# Autodesk Inventor assembly: questionblock
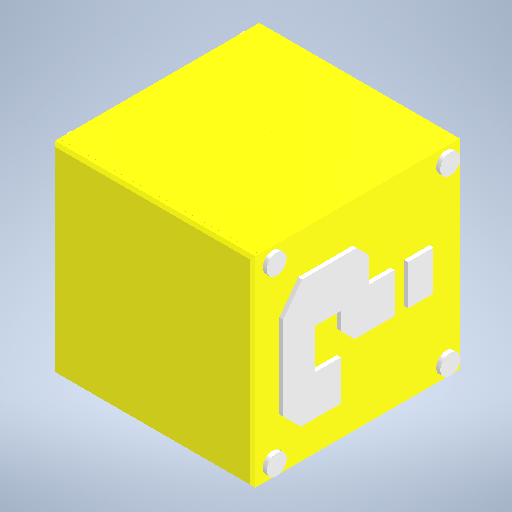
[picture p0: Inventor's stored thumbnail of the model, 512x512]
Saved by Autodesk Inventor 2025 (Build 290162000, 162)
## iProperties
Created: 2024-05-27
Part Number: questionblock
Document SubType Name: Assembly
Designer: wardv
Author: wardv
## Documents named in this file (4)
- C:\Users\wardv\OneDrive\Documents\questionblock.iam
- C:\Users\wardv\OneDrive\Documents\vraagblok.ipt
- C:\Users\wardv\OneDrive\Documents\vraagblok2.ipt
- C:\Users\wardv\OneDrive\Documents\deksel.ipt
## Components (3 placed, 3 different names)
1. vraagblok:1 — Mate:1, Mate:2, Mate:3, Mate:4
2. vraagblok2:1 — Mate:1, Mate:2
3. deksel:1 — Mate:3, Mate:4
## Relationships (4: Mate 4)
- Mate:1: vraagblok:1 ↔ vraagblok2:1
- Mate:2: vraagblok:1 ↔ vraagblok2:1
- Mate:3: vraagblok:1 ↔ deksel:1
- Mate:4: vraagblok:1 ↔ deksel:1
